# Autodesk Inventor assembly: Bluetooth Mount and Board
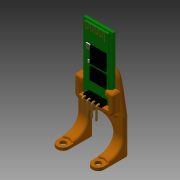
[picture p0: Inventor's stored thumbnail of the model, 180x180]
Saved by Autodesk Inventor 2014 (Build 180170000, 170)
## iProperties
Created: 2014-02-22
Part Number: Bluetooth Mount and Board
Document SubType Name: Assembly
Designer: Spooner
Author: Spooner
## Documents named in this file (3)
- C:\Users\Spooner\Documents\Inventor\FerretBall Robot\3Pod\Inventor 2014 Files\Bluetooth Mount and Board.iam
- C:\Users\Spooner\Documents\Inventor\FerretBall Robot\3Pod\Inventor 2014 Files\Bluetooth Mount.ipt
- C:\Users\Spooner\Documents\Inventor\FerretBall Robot\3Pod\Inventor 2014 Files\JY-MCU Bluetooth Board.ipt
## Components (2 placed, 2 different names)
1. Bluetooth Mount:1 — Mate:1, Mate:2, Mate:3
2. JY-MCU Bluetooth Board:1 — Mate:1, Mate:2, Mate:3
## Relationships (3: Mate 3)
- Mate:1: Bluetooth Mount:1 ↔ JY-MCU Bluetooth Board:1
- Mate:2: Bluetooth Mount:1 ↔ JY-MCU Bluetooth Board:1
- Mate:3 (0.127 mm): Bluetooth Mount:1 ↔ JY-MCU Bluetooth Board:1
